# Autodesk Inventor assembly: ASY Trommel
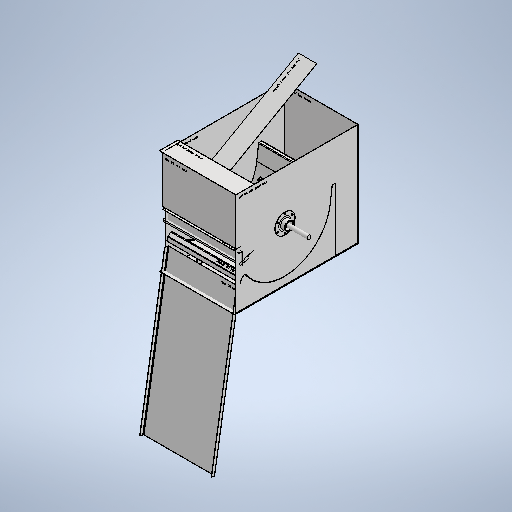
[picture p0: Inventor's stored thumbnail of the model, 512x512]
Saved by Autodesk Inventor 2025 (Build 290162010, 162A)
## iProperties
Created: 2024-08-07
Part Number: ASY Trommel
Document SubType Name: Assembly
Designer: pokla
Author: pokla
## Documents named in this file (23)
- C:\Users\admin\YandexDisk-badmisterfox\домашниий пк\Inventor\BSH_Beshkino_bio_tank\ASY Trommel.iam
- C:\Users\admin\YandexDisk-badmisterfox\домашниий пк\Inventor\BSH_Beshkino_bio_tank\TRM 011 bottom main.ipt
- C:\Users\admin\YandexDisk-badmisterfox\домашниий пк\Inventor\BSH_Beshkino_bio_tank\TRM 012 back main.ipt
- C:\Users\admin\YandexDisk-badmisterfox\домашниий пк\Inventor\BSH_Beshkino_bio_tank\TRM 013 top main.ipt
- C:\Users\admin\YandexDisk-badmisterfox\домашниий пк\Inventor\BSH_Beshkino_bio_tank\TRM 014 face main.ipt
- C:\Users\admin\YandexDisk-badmisterfox\домашниий пк\Inventor\BSH_Beshkino_bio_tank\TRM 015 left board main.ipt
- C:\Users\admin\YandexDisk-badmisterfox\домашниий пк\Inventor\BSH_Beshkino_bio_tank\TRM 017 sheet in.ipt
- C:\Users\admin\YandexDisk-badmisterfox\домашниий пк\Inventor\BSH_Beshkino_bio_tank\TRM 018 clipper.ipt
- C:\Users\admin\YandexDisk-badmisterfox\домашниий пк\Inventor\BSH_Beshkino_bio_tank\TRM 019 tray.ipt
- C:\Users\admin\YandexDisk-badmisterfox\домашниий пк\Inventor\BSH_Beshkino_bio_tank\TRM 021 bottom damper.ipt
- C:\Users\admin\YandexDisk-badmisterfox\домашниий пк\Inventor\BSH_Beshkino_bio_tank\TRM 022 back damper.ipt
- C:\Users\admin\YandexDisk-badmisterfox\домашниий пк\Inventor\BSH_Beshkino_bio_tank\TRM 023 face damper.ipt
- C:\Users\admin\YandexDisk-badmisterfox\домашниий пк\Inventor\BSH_Beshkino_bio_tank\TRM 024 top damper.ipt
- C:\Users\admin\YandexDisk-badmisterfox\домашниий пк\Inventor\BSH_Beshkino_bio_tank\TRM 025 left board damper.ipt
- C:\Users\admin\YandexDisk-badmisterfox\домашниий пк\Inventor\BSH_Beshkino_bio_tank\TRM 026 right board damper.ipt
- C:\Users\admin\YandexDisk-badmisterfox\домашниий пк\Inventor\BSH_Beshkino_bio_tank\TRM 027 tromel.ipt
- C:\Users\admin\YandexDisk-badmisterfox\домашниий пк\Inventor\BSH_Beshkino_bio_tank\TRM 028 main shaft.ipt
- C:\Users\admin\YandexDisk-badmisterfox\домашниий пк\Inventor\BSH_Beshkino_bio_tank\TRM 031 brush.ipt
- C:\Users\admin\YandexDisk-badmisterfox\домашниий пк\Inventor\BSH_Beshkino_bio_tank\TRM 016 right board main+.ipt
- C:\Users\admin\YandexDisk-badmisterfox\домашниий пк\Inventor\BSH_Beshkino_bio_tank\ASY TRM 020 star.iam
- C:\Users\admin\YandexDisk-badmisterfox\домашниий пк\Inventor\BSH_Beshkino_bio_tank\ASY TRM 040 seal.iam
- C:\Users\admin\YandexDisk-badmisterfox\домашниий пк\Inventor\BSH_Beshkino_bio_tank\TRM 032 plate.ipt
- C:\Users\admin\YandexDisk-badmisterfox\домашниий пк\Inventor\BSH_Beshkino_bio_tank\TRM 029 coupling ring.ipt
## Components (23 placed, 22 different names)
1. TRM 011 bottom main:1 — Rigid:25, Mate:11
2. TRM 012 back main:1 — Rigid:22
3. TRM 013 top main:1 — Mate:11
4. TRM 014 face main:1 — Rigid:17
5. TRM 015 left board main:1 — Mate:2, Angle:1, Mate:5, Flush:1, Mate:7, Mate:8, Rigid:17, Rigid:24, Mate:10, Rigid:28
6. TRM 017 sheet in:1 — Rigid:14, Angle:1, Rigid:22
7. TRM 018 clipper:1
8. TRM 019 tray:1
9. TRM 021 bottom damper:1 — Rigid:28, Mate:12
10. TRM 022 back damper:1 — Rigid:24, Rigid:25, Rigid:26
11. TRM 023 face damper:1
12. TRM 024 top damper:1 — Flush:4, Tangent:1, Mate:10
13. TRM 025 left board damper:1 — Mate:12
14. TRM 026 right board damper:1
15. TRM 027 tromel:1 — Rigid:14, Mate:4, Mate:5, Mate:9, Flush:4, Tangent:1
16. TRM 028 main shaft:1 — Mate:1, Mate:2, Mate:4
17. TRM 031 brush:1 — Flush:1, Rigid:21, Flush:3
18. TRM 016 right board main+:1 — Rigid:20, Rigid:26
19. TRM 029 coupling ring:1
20. ASY TRM 020 star:1 [sub-assembly] — Flush:3
21. ASY TRM 040 seal:1 [sub-assembly]
22. ASY TRM 040 seal:2 [sub-assembly] — Rigid:20
23. TRM 032 plate:1 — Rigid:21
## Relationships (29: Mate 12, WeldJoint 11, Flush 4, Angle 1, Tangent 1)
- Rigid:14 [WeldJoint]: TRM 017 sheet in:1 ↔ TRM 027 tromel:1
- Mate:1: TRM 028 main shaft:1
- Mate:2: TRM 015 left board main:1 ↔ TRM 028 main shaft:1
- [Mate]: TRM 028 main shaft:1 ↔ TRM 029 coupling ring:1
- Mate:4: TRM 027 tromel:1 ↔ TRM 028 main shaft:1
- Angle:1 (0 deg): TRM 015 left board main:1 ↔ TRM 017 sheet in:1
- Mate:5: TRM 015 left board main:1 ↔ TRM 027 tromel:1
- Flush:1: TRM 015 left board main:1 ↔ TRM 031 brush:1
- [Mate]: TRM 031 brush:1 ↔ ASY TRM 020 star:1
- [Flush]: TRM 031 brush:1 ↔ ASY TRM 020 star:1
- Mate:7: TRM 015 left board main:1
- Mate:8: TRM 015 left board main:1
- Mate:9: TRM 027 tromel:1
- Rigid:17 [WeldJoint]: TRM 014 face main:1 ↔ TRM 015 left board main:1
- [WeldJoint]: TRM 015 left board main:1 ↔ ASY TRM 040 seal:1
- Rigid:20 [WeldJoint]: TRM 016 right board main+:1 ↔ ASY TRM 040 seal:2
- Rigid:21 [WeldJoint]: TRM 031 brush:1 ↔ TRM 032 plate:1
- Flush:3 (100 mm): TRM 031 brush:1 ↔ ASY TRM 020 star:1
- Rigid:22 [WeldJoint]: TRM 012 back main:1 ↔ TRM 017 sheet in:1
- [WeldJoint]: TRM 029 coupling ring:1 ↔ ASY TRM 020 star:1
- Rigid:24 [WeldJoint]: TRM 015 left board main:1 ↔ TRM 022 back damper:1
- Rigid:25 [WeldJoint]: TRM 011 bottom main:1 ↔ TRM 022 back damper:1
- Flush:4 (5 mm): TRM 024 top damper:1 ↔ TRM 027 tromel:1
- Tangent:1: TRM 024 top damper:1 ↔ TRM 027 tromel:1
- Mate:10: TRM 015 left board main:1 ↔ TRM 024 top damper:1
- Mate:11: TRM 011 bottom main:1 ↔ TRM 013 top main:1
- Rigid:26 [WeldJoint]: TRM 022 back damper:1 ↔ TRM 016 right board main+:1
- Rigid:28 [WeldJoint]: TRM 015 left board main:1 ↔ TRM 021 bottom damper:1
- Mate:12: TRM 021 bottom damper:1 ↔ TRM 025 left board damper:1
